# Autodesk Inventor assembly: Thumb Screw Assy
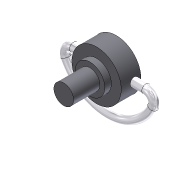
[picture p0: Inventor's stored thumbnail of the model, 180x180]
Saved by Autodesk Inventor 2011 (Build 150239000, 239)
## iProperties
Created: 2012-10-13
Part Number: Thumb Screw Assy
Document SubType Name: Assembly
Designer: Lance
Author: Lance
## Documents named in this file (3)
- C:\Inventor Projects\MPX0032 - Projector Accessories\Manfrotto 494RC2 - Tripod Head\Thumb Screw Assy.iam
- C:\Inventor Projects\MPX0032 - Projector Accessories\Manfrotto 494RC2 - Tripod Head\Thumb Screw.ipt
- C:\Inventor Projects\MPX0032 - Projector Accessories\Manfrotto 494RC2 - Tripod Head\Thumb Screw Handle.ipt
## Components (2 placed, 2 different names)
1. Thumb Screw:1 — Flush:1, Angle:1, Mate:1
2. Thumb Screw Handle:1 — Flush:1, Angle:1, Mate:1
## Relationships (3: Flush 1, Angle 1, Mate 1)
- Flush:1: Thumb Screw:1 ↔ Thumb Screw Handle:1
- Angle:1 (0 deg): Thumb Screw:1 ↔ Thumb Screw Handle:1
- Mate:1: Thumb Screw:1 ↔ Thumb Screw Handle:1
